# Autodesk Inventor assembly: 2f2
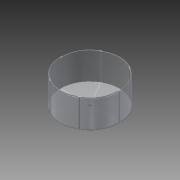
[picture p0: Inventor's stored thumbnail of the model, 180x180]
Saved by Autodesk Inventor 2014 (Build 180170000, 170)
## iProperties
Company: HERA Project
Created: 2013-06-27
Part Number: 2f2
Document SubType Name: Assembly
Designer: David DeBoer
Description: Feed backplane support assembly
Author: David DeBoer
Title: Feed backplane support
## Documents named in this file (9)
- C:\Users\ddeboer\Desktop\hera-cad\feed\bpScreenAssembly.iam
- C:\Users\ddeboer\Desktop\hera-cad\feed\bpSupArm.ipt
- C:\Users\ddeboer\Desktop\hera-cad\smallParts\pvc_T_0.75in.ipt
- C:\Users\ddeboer\Desktop\hera-cad\feed\bpSupArc.ipt
- C:\Users\ddeboer\Desktop\hera-cad\feed\bpScreen.ipt
- C:\Users\ddeboer\Desktop\hera-cad\feed\bpCylinder.ipt
- C:\Users\ddeboer\Desktop\hera-cad\jigs\bpSparJig.ipt
- C:\Users\ddeboer\Desktop\hera-cad\feed\bpSupVertArm.ipt
- C:\Users\ddeboer\Desktop\hera-cad\smallParts\angleBracketB.ipt
## Components (45 placed, 8 different names)
1. bpSparJig:1 — Insert:6, Insert:7, Insert:8
2. bpScreen:1 — Insert:8, Angle:3, Insert:13
3. bpCylinder:1 — Insert:13
4. bpSupArm:1 — Insert:4, Angle:1, Angle:2, Insert:6, Insert:7, Angle:9
5. pvc_T_0.75in:1 — Insert:4, Insert:5, Angle:2, Insert:16
6. bpSupArc:1 — Insert:5, Angle:1
7. bpSupArm:2
8. pvc_T_0.75in:2 — Angle:10
9. bpSupArc:2
10. bpSupArm:3
11. pvc_T_0.75in:3 — Angle:3
12. bpSupArc:3
13. bpSupArm:4
14. pvc_T_0.75in:4
15. bpSupArc:4
16. bpSupArm:5
17. pvc_T_0.75in:5
18. bpSupArc:5
19. bpSupArm:6
20. pvc_T_0.75in:6
21. bpSupArc:6
22. angleBracketB:1 — Insert:14, Insert:15, Angle:8, Angle:9, Insert:16
23. bpSupVertArm:1 — Insert:11, Insert:14, Insert:15
24. pvc_T_0.75in:7 — Insert:11, Insert:12, Angle:8
25. bpSupArc:7 — Insert:12, Angle:10
26. angleBracketB:2
27. bpSupVertArm:2
28. pvc_T_0.75in:8
29. bpSupArc:8
30. angleBracketB:3
31. bpSupVertArm:3
32. pvc_T_0.75in:9
33. bpSupArc:9
34. angleBracketB:4
35. bpSupVertArm:4
36. pvc_T_0.75in:10
37. bpSupArc:10
38. angleBracketB:5
39. bpSupVertArm:5
40. pvc_T_0.75in:11
41. bpSupArc:11
42. angleBracketB:6
43. bpSupVertArm:6
44. pvc_T_0.75in:12
45. bpSupArc:12
## Component patterns: (6 elements, first: bpSupArm:1 + pvc_T_0.75in:1 + bpSupArc:1), (6 elements, first: angleBracketB:1 + bpSupVertArm:1 + pvc_T_0.75in:7 + bpSupArc:7)
## Relationships (17: Insert 11, Angle 6)
- Insert:4 (-12.7 mm): bpSupArm:1 ↔ pvc_T_0.75in:1
- Insert:5: pvc_T_0.75in:1 ↔ bpSupArc:1
- Angle:1 (30 deg): bpSupArm:1 ↔ bpSupArc:1
- Angle:2 (90 deg): bpSupArm:1 ↔ pvc_T_0.75in:1
- Insert:6: bpSparJig:1 ↔ bpSupArm:1
- Insert:7: bpSparJig:1 ↔ bpSupArm:1
- Insert:8 (25.4 mm): bpSparJig:1 ↔ bpScreen:1
- Angle:3 (180 deg): bpScreen:1 ↔ pvc_T_0.75in:3
- Insert:11 (-12.7 mm): bpSupVertArm:1 ↔ pvc_T_0.75in:7
- Insert:12 (-12.7 mm): pvc_T_0.75in:7 ↔ bpSupArc:7
- Insert:13: bpScreen:1 ↔ bpCylinder:1
- Insert:14: angleBracketB:1 ↔ bpSupVertArm:1
- Insert:15: angleBracketB:1 ↔ bpSupVertArm:1
- Angle:8 (90 deg): angleBracketB:1 ↔ pvc_T_0.75in:7
- Angle:9 (0 deg): bpSupArm:1 ↔ angleBracketB:1
- Insert:16: pvc_T_0.75in:1 ↔ angleBracketB:1
- Angle:10 (0 deg): pvc_T_0.75in:2 ↔ bpSupArc:7
